# Autodesk Inventor assembly: KONARM_CALY
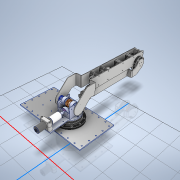
[picture p0: Inventor's stored thumbnail of the model, 180x180]
Saved by Autodesk Inventor 2022 (Build 260153000, 153)
## iProperties
Created: 2023-01-29
Part Number: KONARM_CALY
Document SubType Name: Assembly
Designer: Kamil
Author: Kamil
## Documents named in this file (6)
- D:\konarm 3 przegub\KONARM_CALY.iam
- D:\konarm 3 przegub\Konarm_3_przegub_v2.iam
- C:\Users\Kamil\Downloads\Złożenie2.STEP.ipt
- D:\Konarm_1_przegub_final\I_Przegub_final.iam
- D:\konarm 3 przegub\Uchwyt_silnika_KONARM_3.ipt
- D:\KONARM\Konarm_1_przegub_final\Uchwyt_silnika_2_dół.ipt
## Components (5 placed, 5 different names)
1. Konarm_3_przegub_v2:1 [sub-assembly] — Mate:4, Mate:5
2. Złożenie2.STEP:1 — Mate:1, Mate:2, Mate:4, Mate:5, Mate:6, Mate:7, Mate:8, Mate:9
3. I_Przegub_final:1 [sub-assembly] — Mate:1, Mate:2
4. Uchwyt_silnika_KONARM_3:1 — Mate:6, Mate:7, Mate:8, Mate:10
5. Uchwyt_silnika_2_dół:1 — Mate:9, Mate:10
## Relationships (9: Mate 9)
- Mate:1: Złożenie2.STEP:1 ↔ I_Przegub_final:1
- Mate:2: Złożenie2.STEP:1 ↔ I_Przegub_final:1
- Mate:4: Konarm_3_przegub_v2:1 ↔ Złożenie2.STEP:1
- Mate:5: Konarm_3_przegub_v2:1 ↔ Złożenie2.STEP:1
- Mate:6: Złożenie2.STEP:1 ↔ Uchwyt_silnika_KONARM_3:1
- Mate:7: Złożenie2.STEP:1 ↔ Uchwyt_silnika_KONARM_3:1
- Mate:8: Złożenie2.STEP:1 ↔ Uchwyt_silnika_KONARM_3:1
- Mate:9: Złożenie2.STEP:1 ↔ Uchwyt_silnika_2_dół:1
- Mate:10: Uchwyt_silnika_KONARM_3:1 ↔ Uchwyt_silnika_2_dół:1
